# Autodesk Inventor assembly: Screw_Joint_36T_Custom_Spacer
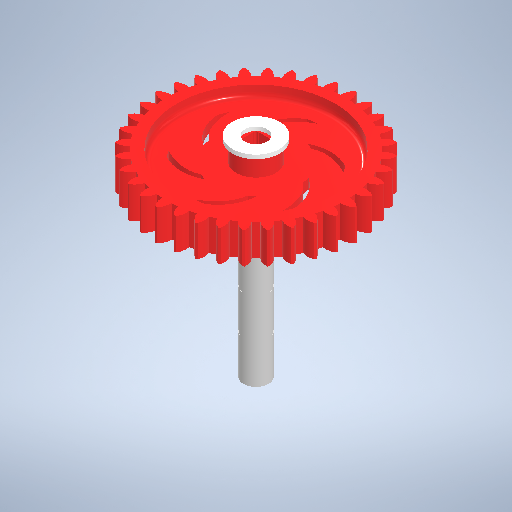
[picture p0: Inventor's stored thumbnail of the model, 512x512]
Saved by Autodesk Inventor 2025 (Build 290162000, 162)
## iProperties
Created: 2024-12-08
Part Number: Screw_Joint_36T_Custom_Spacer
Document SubType Name: Assembly
Designer: Aditya Koduri
Author: Aditya Koduri
## Documents named in this file (5)
- C:\Users\mzart\Downloads\Full_Cad_Model\Screw_Joint_36T_Custom_Spacer.iam
- C:\Users\mzart\Downloads\VEX-CAD-Inventor-main\VEX-CAD-Inventor-main\Motion\Spacers\Washer Teflon\TWasher .375 OD x .03125.ipt
- C:\Users\mzart\Downloads\VEX-CAD-Inventor-main\VEX-CAD-Inventor-main\Motion\Gears\LS 36T Gear.ipt
- C:\Users\mzart\Downloads\Full_Cad_Model\Thin_spacer_custom.ipt
- C:\Users\mzart\Downloads\VEX-CAD-Inventor-main\VEX-CAD-Inventor-main\Motion\Spacers\Washer Teflon.ipt
## Components (6 placed, 3 different names)
1. TWasher .375 OD x .03125:1
2. LS 36T Gear:1
3. Thin_spacer_custom:1
4. Thin_spacer_custom:2
5. Thin_spacer_custom:3
6. Thin_spacer_custom:4
## Relationships (5: Insert 5)
- [Insert]: TWasher .375 OD x .03125:1 ↔ LS 36T Gear:1
- [Insert]: Thin_spacer_custom:1 ↔ Thin_spacer_custom:3
- [Insert]: Thin_spacer_custom:1 ↔ Thin_spacer_custom:4
- [Insert]: Thin_spacer_custom:2 ↔ Thin_spacer_custom:3
- [Insert]: LS 36T Gear:1 ↔ Thin_spacer_custom:2
